# Autodesk Inventor assembly: RemoteCameraModule
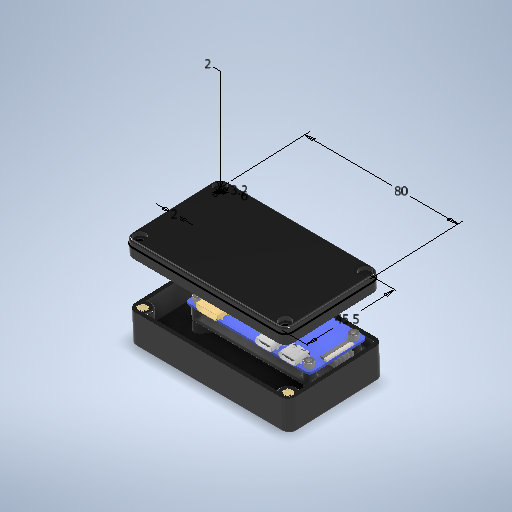
[picture p0: Inventor's stored thumbnail of the model, 512x512]
Saved by Autodesk Inventor 2025 (Build 290162000, 162)
## iProperties
Created: 2025-02-27
Part Number: RemoteCameraModule
Document SubType Name: Assembly
Designer: tvoko
Author: tvoko
## Documents named in this file (10)
- D:\github\enhanced-radio-comm\demo-hardware\RemoteCameraModule.iam
- C:\Users\tvoko\Documents\School\Fall 2024\Senior Design Pt 1\Lab 1\Buyouts\OPiZ2W_\OPiZ2W_.ipt
- D:\github\enhanced-radio-comm\demo-hardware\PiMountBracket.ipt
- D:\github\enhanced-radio-comm\demo-hardware\RemoteCasing.ipt
- C:\Users\tvoko\Documents\School\Fall 2024\Senior Design Pt 1\Lab 1\Buyouts\Arducam USB Camera module B0431\Arducam USB Camera module B0431.ipt
- C:\Users\tvoko\Documents\Inventor\Content Center Files\R2025\en-US\IS 2269\IS 2269 - M2.5 x 12.ipt
- D:\github\enhanced-radio-comm\demo-hardware\RemoteCasingBackCover.ipt
- C:\Users\tvoko\Documents\School\Fall 2024\Senior Design Pt 1\Lab 1\Buyouts\Insert M3 D5 L5mm\Insert M3 D5 L5mm.ipt
- D:\github\enhanced-radio-comm\demo-hardware\HEATSINK14x14.ipt
- D:\github\enhanced-radio-comm\demo-hardware\HEATSINK9x9.ipt
## Components (14 placed, 9 different names)
1. OPiZ2W_:1 — Mate:1, Mate:2, Mate:8, Mate:10, Mate:12, Mate:14, Mate:24, Flush:4, Flush:5, Mate:32, Mate:34
2. PiMountBracket:1 — Mate:1, Mate:2, Mate:4, Mate:9, Mate:11, Mate:13, Mate:20, Mate:21, Mate:22, Mate:23, Mate:24, Mate:25
3. IS 2269 M2.5 x 12:1 — Mate:4, Mate:8
4. IS 2269 M2.5 x 12:2 — Mate:9, Mate:10
5. IS 2269 M2.5 x 12:3 — Mate:11, Mate:12
6. IS 2269 M2.5 x 12:4 — Mate:13, Mate:14
7. RemoteCasing:1 — Mate:17, Mate:18, Mate:19, Mate:20, Mate:21, Mate:22, Mate:23, Mate:25, Mate:26, Mate:27, Mate:28, Flush:1, Flush:2, Flush:3, Mate:29, Mate:30, Mate:31
8. Arducam USB Camera module B0431:1 — Mate:17, Mate:18, Mate:19
9. RemoteCasingBackCover:1 — Mate:29, Mate:30, Mate:31
10. Insert M3 D5 L5mm:1 — Mate:26, Flush:1
11. Insert M3 D5 L5mm:2 — Mate:27, Flush:2
12. Insert M3 D5 L5mm:3 — Mate:28, Flush:3
13. HEATSINK14x14:1 — Flush:4, Flush:5, Mate:32, Mate:33, Flush:6
14. HEATSINK9x9:1 — Mate:33, Mate:34, Flush:6
## Relationships (34: Mate 28, Flush 6)
- Mate:1: OPiZ2W_:1 ↔ PiMountBracket:1
- Mate:2: OPiZ2W_:1 ↔ PiMountBracket:1
- Mate:4: PiMountBracket:1 ↔ IS 2269 M2.5 x 12:1
- Mate:8: OPiZ2W_:1 ↔ IS 2269 M2.5 x 12:1
- Mate:9: PiMountBracket:1 ↔ IS 2269 M2.5 x 12:2
- Mate:10: OPiZ2W_:1 ↔ IS 2269 M2.5 x 12:2
- Mate:11: PiMountBracket:1 ↔ IS 2269 M2.5 x 12:3
- Mate:12: OPiZ2W_:1 ↔ IS 2269 M2.5 x 12:3
- Mate:13: PiMountBracket:1 ↔ IS 2269 M2.5 x 12:4
- Mate:14: OPiZ2W_:1 ↔ IS 2269 M2.5 x 12:4
- Mate:17: RemoteCasing:1 ↔ Arducam USB Camera module B0431:1
- Mate:18: RemoteCasing:1 ↔ Arducam USB Camera module B0431:1
- Mate:19: RemoteCasing:1 ↔ Arducam USB Camera module B0431:1
- Mate:20: PiMountBracket:1 ↔ RemoteCasing:1
- Mate:21: PiMountBracket:1 ↔ RemoteCasing:1
- Mate:22: PiMountBracket:1 ↔ RemoteCasing:1
- Mate:23: PiMountBracket:1 ↔ RemoteCasing:1
- Mate:24: OPiZ2W_:1 ↔ PiMountBracket:1
- Mate:25: PiMountBracket:1 ↔ RemoteCasing:1
- Mate:26: RemoteCasing:1 ↔ Insert M3 D5 L5mm:1
- Mate:27: RemoteCasing:1 ↔ Insert M3 D5 L5mm:2
- Mate:28: RemoteCasing:1 ↔ Insert M3 D5 L5mm:3
- Flush:1: RemoteCasing:1 ↔ Insert M3 D5 L5mm:1
- Flush:2: RemoteCasing:1 ↔ Insert M3 D5 L5mm:2
- Flush:3: RemoteCasing:1 ↔ Insert M3 D5 L5mm:3
- Mate:29: RemoteCasing:1 ↔ RemoteCasingBackCover:1
- Mate:30: RemoteCasing:1 ↔ RemoteCasingBackCover:1
- Mate:31: RemoteCasing:1 ↔ RemoteCasingBackCover:1
- Flush:4: OPiZ2W_:1 ↔ HEATSINK14x14:1
- Flush:5: OPiZ2W_:1 ↔ HEATSINK14x14:1
- Mate:32: OPiZ2W_:1 ↔ HEATSINK14x14:1
- Mate:33: HEATSINK14x14:1 ↔ HEATSINK9x9:1
- Mate:34: OPiZ2W_:1 ↔ HEATSINK9x9:1
- Flush:6: HEATSINK14x14:1 ↔ HEATSINK9x9:1
